# Autodesk Inventor assembly: ASY Trommel
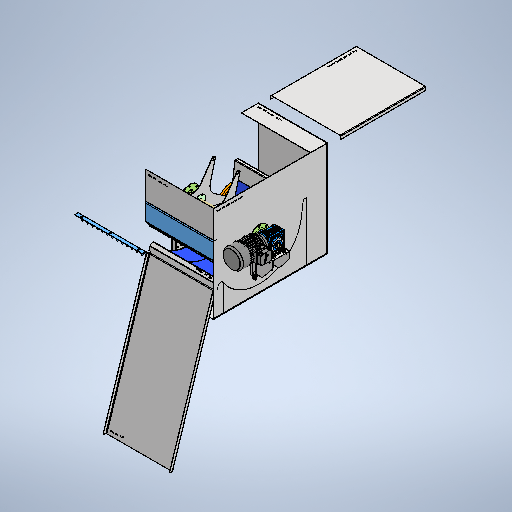
[picture p0: Inventor's stored thumbnail of the model, 512x512]
Saved by Autodesk Inventor 2025.1 (Build 291241020, 241B)
## iProperties
Created: 2024-08-07
Part Number: ASY Trommel
Document SubType Name: Assembly
Designer: pokla
Mass: 80063.4 g
Surface Area: 94462 cm^2
Volume: 14055.1 cm^3
Density: 5.6964 g/cm^3
Author: pokla
## Documents named in this file (31)
- C:\Users\user\YandexDisk-badmisterfox\домашниий пк\Inventor\BSH_Beshkino_bio_tank\ASY Trommel.iam
- C:\Users\user\YandexDisk-badmisterfox\домашниий пк\Inventor\BSH_Beshkino_bio_tank\TRM 011 bottom main.ipt
- C:\Users\user\YandexDisk-badmisterfox\домашниий пк\Inventor\BSH_Beshkino_bio_tank\TRM 012 back main.ipt
- C:\Users\user\YandexDisk-badmisterfox\домашниий пк\Inventor\BSH_Beshkino_bio_tank\TRM 013 top main.ipt
- C:\Users\user\YandexDisk-badmisterfox\домашниий пк\Inventor\BSH_Beshkino_bio_tank\TRM 014 face main.ipt
- C:\Users\user\YandexDisk-badmisterfox\домашниий пк\Inventor\BSH_Beshkino_bio_tank\TRM 015 left board main.ipt
- C:\Users\user\YandexDisk-badmisterfox\домашниий пк\Inventor\BSH_Beshkino_bio_tank\TRM 017 sheet in.ipt
- C:\Users\user\YandexDisk-badmisterfox\домашниий пк\Inventor\BSH_Beshkino_bio_tank\TRM 018 clipper.ipt
- C:\Users\user\YandexDisk-badmisterfox\домашниий пк\Inventor\BSH_Beshkino_bio_tank\TRM 019 tray.ipt
- C:\Users\user\YandexDisk-badmisterfox\домашниий пк\Inventor\BSH_Beshkino_bio_tank\TRM 021 bottom damper.ipt
- C:\Users\user\YandexDisk-badmisterfox\домашниий пк\Inventor\BSH_Beshkino_bio_tank\TRM 022 back damper.ipt
- C:\Users\user\YandexDisk-badmisterfox\домашниий пк\Inventor\BSH_Beshkino_bio_tank\TRM 023 face damper.ipt
- C:\Users\user\YandexDisk-badmisterfox\домашниий пк\Inventor\BSH_Beshkino_bio_tank\TRM 024 top damper.ipt
- C:\Users\user\YandexDisk-badmisterfox\домашниий пк\Inventor\BSH_Beshkino_bio_tank\TRM 025 left board damper.ipt
- C:\Users\user\YandexDisk-badmisterfox\домашниий пк\Inventor\BSH_Beshkino_bio_tank\TRM 027 tromel.ipt
- C:\Users\user\YandexDisk-badmisterfox\домашниий пк\Inventor\BSH_Beshkino_bio_tank\TRM 031 brush.ipt
- C:\Users\user\YandexDisk-badmisterfox\домашниий пк\Inventor\BSH_Beshkino_bio_tank\ASY TRM 020 star.iam
- C:\Users\user\YandexDisk-badmisterfox\домашниий пк\Inventor\BSH_Beshkino_bio_tank\TRM 032 plate.ipt
- C:\Users\user\YandexDisk-badmisterfox\домашниий пк\Inventor\BSH_Beshkino_bio_tank\TRM 016 right board main++.ipt
- C:\Users\user\YandexDisk-badmisterfox\домашниий пк\Inventor\BSH_Beshkino_bio_tank\3d party\motor-reductor NMRV040\motor-reductor NMRV040.iam
- C:\Users\user\YandexDisk-badmisterfox\домашниий пк\Inventor\BSH_Beshkino_bio_tank\TRM 036 box 1.ipt
- C:\Users\user\YandexDisk-badmisterfox\домашниий пк\Inventor\BSH_Beshkino_bio_tank\TRM 037 box 2.ipt
- C:\Users\user\YandexDisk-badmisterfox\домашниий пк\Inventor\BSH_Beshkino_bio_tank\TRM 038 facr wall.ipt
- C:\Users\user\YandexDisk-badmisterfox\домашниий пк\Inventor\BSH_Beshkino_bio_tank\ASY TRM 050 shaft.iam
- C:\Users\user\YandexDisk-badmisterfox\домашниий пк\Inventor\BSH_Beshkino_bio_tank\Assembly1.iam
- C:\Users\user\YandexDisk-badmisterfox\домашниий пк\Inventor\BSH_Beshkino_bio_tank\3d party\Stamp flange DIN2642\Stamd flange lapped collar DIN2642\Stamp flange DIN2642-080.ipt
- C:\Users\user\YandexDisk-badmisterfox\домашниий пк\Inventor\BSH_Beshkino_bio_tank\3d party\Stamp flange DIN2642\Stamd flange lapped collar DIN2642.ipt
- C:\Users\user\YandexDisk-badmisterfox\домашниий пк\Inventor\BSH_Beshkino_bio_tank\3d party\MSC 105 rocket tube 9.ipt
- C:\Users\user\YandexDisk-badmisterfox\домашниий пк\Inventor\BSH_Beshkino_bio_tank\TRM 030 star conrtforce plate.ipt
- C:\Users\user\YandexDisk-badmisterfox\домашниий пк\Inventor\BSH_Beshkino_bio_tank\TRM 018 comb 2.ipt
- C:\Users\user\YandexDisk-badmisterfox\домашниий пк\Inventor\BSH_Beshkino_bio_tank\TRM 34 comb 3.ipt
## Components (37 placed, 30 different names)
1. TRM 011 bottom main:1 — Rigid:25, Mate:11, Mate:23, Flush:7, Rigid:43, Rigid:45
2. TRM 012 back main:1 — Rigid:22, Mate:12
3. TRM 013 top main:1 — Mate:11, Mate:12, Rigid:33
4. TRM 014 face main:1 — Rigid:17, Slider:2
5. TRM 015 left board main:1 — Angle:1, Mate:5, Flush:1, Mate:7, Mate:8, Rigid:17, Rotational:20, Rigid:24, Mate:10, Rigid:28, Angle:2, Mate:16, Mate:24
6. TRM 016 right board main++:1 — Rigid:29, Rotational:31, Rigid:32, Mate:20, Mate:21, Rigid:42, Rigid:44
7. TRM 017 sheet in:1 — Rigid:14, Angle:1, Rigid:22
8. TRM 018 clipper:1 — Slider:2, Angle:4, Slider:3
9. TRM 019 tray:1 — Mate:13, Mate:14
10. TRM 021 bottom damper:1 — Rigid:28
11. TRM 022 back damper:1 — Rigid:24, Rigid:25, Rigid:29
12. TRM 023 face damper:1 — Mate:16, Rigid:34
13. TRM 024 top damper:1 — Flush:4, Mate:10, Tangent:1, Mate:13
14. TRM 027 tromel:1 — Rigid:14, Mate:5, Mate:9, Flush:4, Tangent:1
15. TRM 031 brush:1 — Flush:1, Angle:4
16. ASY TRM 020 star:1 [sub-assembly] — Rigid:50
17. ASY TRM 050 shaft:1 [sub-assembly] — Rigid:50, Rotational:20, Rotational:31, Rigid:47, Rigid:49
18. TRM 032 plate:1 — Rigid:48
19. TRM 021 bottom damper:2 — Rigid:32, Mate:19, Mate:22
20. TRM 025 left board damper:2 — Mate:19, Mate:22
21. TRM 013 top main:2 — Rigid:33
22. ASY TRM 020 star:2 [sub-assembly] — Rigid:49, Rigid:51
23. motor-reductor NMRV040:1 [sub-assembly] — Angle:2, Mate:25
24. 023 TRM face damper:2 — Rigid:34, Flush:7
25. ASY TRM 020 star:3 [sub-assembly] — Rigid:47, Rigid:48
26. TRM 036 box 1:1 — Rigid:38
27. TRM 037 box 2:1 — Mate:20, Mate:21, Rigid:38, Rigid:39
28. TRM 036 box 1:2 — Rigid:39
29. TRM 038 facr wall:1 — Mate:23, Mate:24
30. Assembly1:1 [sub-assembly] — Mate:25
31. Stamp flange DIN2642-080:1 — Rigid:42
32. Stamp flange DIN2642-080:2 — Rigid:43
33. MSC 105 rocket tube 9:1 — Rigid:44
34. MSC 105 rocket tube 9:2 — Rigid:45
35. TRM 030 star conrtforce plate:1 — Rigid:51
36. TRM 018 comb 2:1 — Slider:3
37. TRM 34 comb 3:1
## Relationships (58: Mate 23, WeldJoint 21, Angle 4, Flush 4, TranslationJoint 3, RevoluteJoint 2, Tangent 1)
- Rigid:14 [WeldJoint]: TRM 017 sheet in:1 ↔ TRM 027 tromel:1
- [Mate]: ASY TRM 050 shaft:1
- [Mate]: TRM 015 left board main:1 ↔ ASY TRM 050 shaft:1
- [Mate]: TRM 027 tromel:1 ↔ ASY TRM 050 shaft:1
- Angle:1 (0 deg): TRM 015 left board main:1 ↔ TRM 017 sheet in:1
- Mate:5: TRM 015 left board main:1 ↔ TRM 027 tromel:1
- Flush:1 (2 mm): TRM 015 left board main:1 ↔ TRM 031 brush:1
- [Mate]: TRM 031 brush:1 ↔ ASY TRM 020 star:1
- [Flush]: TRM 031 brush:1 ↔ ASY TRM 020 star:1
- Mate:7: TRM 015 left board main:1
- Mate:8: TRM 015 left board main:1
- Mate:9: TRM 027 tromel:1
- Rigid:17 [WeldJoint]: TRM 014 face main:1 ↔ TRM 015 left board main:1
- Rotational:20 [RevoluteJoint]: TRM 015 left board main:1 ↔ ASY TRM 050 shaft:1
- Rigid:22 [WeldJoint]: TRM 012 back main:1 ↔ TRM 017 sheet in:1
- Rigid:50 [WeldJoint]: ASY TRM 020 star:1 ↔ ASY TRM 050 shaft:1
- Rigid:24 [WeldJoint]: TRM 015 left board main:1 ↔ TRM 022 back damper:1
- Rigid:25 [WeldJoint]: TRM 011 bottom main:1 ↔ TRM 022 back damper:1
- Flush:4 (15 mm): TRM 024 top damper:1 ↔ TRM 027 tromel:1
- Mate:10: TRM 015 left board main:1 ↔ TRM 024 top damper:1
- Tangent:1: TRM 024 top damper:1 ↔ TRM 027 tromel:1
- Rigid:28 [WeldJoint]: TRM 015 left board main:1 ↔ TRM 021 bottom damper:1
- Rigid:29 [WeldJoint]: TRM 016 right board main++:1 ↔ TRM 022 back damper:1
- Rotational:31 [RevoluteJoint]: TRM 016 right board main++:1 ↔ ASY TRM 050 shaft:1
- Rigid:32 [WeldJoint]: TRM 016 right board main++:1 ↔ TRM 021 bottom damper:2
- Mate:11: TRM 011 bottom main:1 ↔ TRM 013 top main:1
- Mate:12: TRM 012 back main:1 ↔ TRM 013 top main:1
- Mate:13: TRM 019 tray:1 ↔ TRM 024 top damper:1
- Mate:14: TRM 019 tray:1
- Rigid:33 [WeldJoint] (200 mm): TRM 013 top main:1 ↔ TRM 013 top main:2
- [Mate]: ASY TRM 050 shaft:1 ↔ motor-reductor NMRV040:1
- Angle:2 (0 deg): TRM 015 left board main:1 ↔ motor-reductor NMRV040:1
- Mate:16: TRM 015 left board main:1 ↔ TRM 023 face damper:1
- [TranslationJoint]: 023 TRM face damper:2 ↔ Assembly1:1
- [Mate]: ASY TRM 050 shaft:1 ↔ Assembly1:1
- Rigid:34 [WeldJoint] (120 mm): TRM 023 face damper:1 ↔ 023 TRM face damper:2
- [Angle] (0 deg): TRM 011 bottom main:1 ↔ Assembly1:1
- Mate:19: TRM 021 bottom damper:2 ↔ TRM 025 left board damper:2
- Mate:20: TRM 016 right board main++:1 ↔ TRM 037 box 2:1
- Mate:21 (-2 mm): TRM 016 right board main++:1 ↔ TRM 037 box 2:1
- Rigid:38 [WeldJoint]: TRM 036 box 1:1 ↔ TRM 037 box 2:1
- Rigid:39 [WeldJoint]: TRM 037 box 2:1 ↔ TRM 036 box 1:2
- Mate:22: TRM 021 bottom damper:2 ↔ TRM 025 left board damper:2
- Mate:23: TRM 011 bottom main:1 ↔ TRM 038 facr wall:1
- Mate:24: TRM 015 left board main:1 ↔ TRM 038 facr wall:1
- Mate:25: motor-reductor NMRV040:1 ↔ Assembly1:1
- Flush:7 (140 mm): TRM 011 bottom main:1 ↔ 023 TRM face damper:2
- Rigid:42 [WeldJoint] (100 mm): TRM 016 right board main++:1 ↔ Stamp flange DIN2642-080:1
- Rigid:43 [WeldJoint] (-100 mm): TRM 011 bottom main:1 ↔ Stamp flange DIN2642-080:2
- Rigid:44 [WeldJoint]: TRM 016 right board main++:1 ↔ MSC 105 rocket tube 9:1
- Rigid:45 [WeldJoint]: TRM 011 bottom main:1 ↔ MSC 105 rocket tube 9:2
- Rigid:47 [WeldJoint]: ASY TRM 050 shaft:1 ↔ ASY TRM 020 star:3
- Rigid:49 [WeldJoint]: ASY TRM 050 shaft:1 ↔ ASY TRM 020 star:2
- Rigid:48 [WeldJoint]: TRM 032 plate:1 ↔ ASY TRM 020 star:3
- Rigid:51 [WeldJoint]: ASY TRM 020 star:2 ↔ TRM 030 star conrtforce plate:1
- Slider:2 [TranslationJoint]: TRM 014 face main:1 ↔ TRM 018 clipper:1
- Angle:4 (0 deg): TRM 018 clipper:1 ↔ TRM 031 brush:1
- Slider:3 [TranslationJoint]: TRM 018 clipper:1 ↔ TRM 018 comb 2:1
